# Autodesk Inventor assembly: Doppia Giuntura
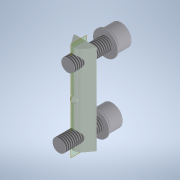
[picture p0: Inventor's stored thumbnail of the model, 180x180]
Saved by Autodesk Inventor 2022 (Build 260153000, 153)
## iProperties
Created: 2021-12-29
Part Number: Doppia Giuntura
Document SubType Name: Assembly
Designer: matte
Author: matte
## Documents named in this file (4)
- C:\Users\matte\Documents\GitHub\MDM-CyberOrto-CAD\Pezzi singoli\Supporto lineare\Doppia Giuntura.iam
- C:\Users\matte\Documents\GitHub\MDM-CyberOrto-CAD\Parker components\02-Fasteners\15-T-Bolts_Nuts_Washers\03-Washers\24-708-8.ipt
- C:\Users\matte\Documents\GitHub\MDM-CyberOrto-CAD\Parker components\02-Fasteners\16-Screws\01-Metric Screws\03-Socket Head\24-325-8.ipt
- C:\Users\matte\Documents\GitHub\MDM-CyberOrto-CAD\Parker components\02-Fasteners\10-Standard T-Nuts\20-050.ipt
## Components (5 placed, 3 different names)
1. 24-708-8:1
2. 24-325-8:1 — Coincidente:9
3. 24-708-8:2 — Coincidente:7
4. 24-325-8:2 — Coincidente:8
5. 20-050:1 — Coincidente:7, Coincidente:8, Coincidente:9
## Relationships (7: Mate 7)
- [Mate]: 24-708-8:1 ↔ 24-325-8:1
- [Mate] (1 mm): 24-708-8:1 ↔ 24-325-8:1
- [Mate]: 24-708-8:2 ↔ 24-325-8:2
- [Mate] (1 mm): 24-708-8:2 ↔ 24-325-8:2
- Coincidente:7 [Mate] (12 mm): 24-708-8:2 ↔ 20-050:1
- Coincidente:8 [Mate]: 24-325-8:2 ↔ 20-050:1
- Coincidente:9 [Mate]: 24-325-8:1 ↔ 20-050:1
## Named parameters: d4_d28 = 0 mm, d5_d29 = 1 mm
